# Autodesk Inventor assembly: Cover Optical Camera Only
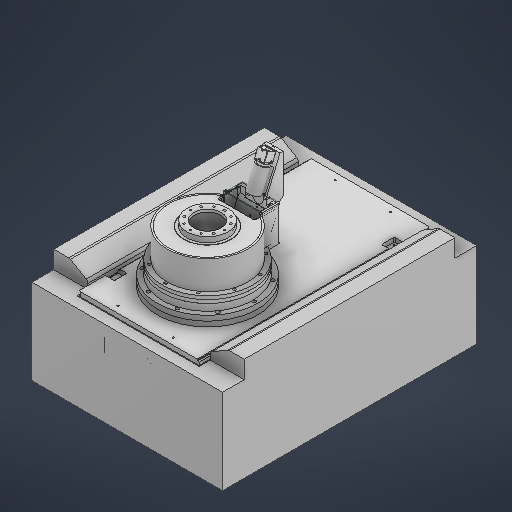
[picture p0: Inventor's stored thumbnail of the model, 512x512]
Saved by Autodesk Inventor 2025 (Build 290162000, 162)
## iProperties
Created: 2025-02-04
Part Number: Cover Optical Camera Only
Document SubType Name: Assembly
Designer: mayhe
Author: mayhe
## Documents named in this file (18)
- C:\Users\mayhe\OneDrive\Documents\GitHub\In-situ-monitoring-of-powder-bed-fusion-additive-manufacturing\system_development\Mithril\v0.2\Model\Cover Optical Camera Only.iam
- C:\Users\mayhe\OneDrive\Documents\GitHub\In-situ-monitoring-of-powder-bed-fusion-additive-manufacturing\system_development\Mithril\v0.2\Model\Cover (Optical Camera).ipt
- C:\Users\mayhe\OneDrive\Documents\GitHub\In-situ-monitoring-of-powder-bed-fusion-additive-manufacturing\system_development\Mithril\v0.2\Model\300mm Housing 1.ipt
- C:\Users\mayhe\OneDrive\Documents\GitHub\In-situ-monitoring-of-powder-bed-fusion-additive-manufacturing\system_development\Mithril\v0.2\Model\Cylinder Spacer Optical Camera.ipt
- C:\Users\mayhe\OneDrive\Documents\GitHub\In-situ-monitoring-of-powder-bed-fusion-additive-manufacturing\system_development\Mithril\v0.2\Model\Cylinder Segment\Cylinder Slidey Bit Housings\Cylinder Slidey Bit Housing Camera only v0.2.ipt
- C:\Users\mayhe\OneDrive\Documents\GitHub\In-situ-monitoring-of-powder-bed-fusion-additive-manufacturing\system_development\Mithril\v0.2\Model\300mm housing 2 Camera.ipt
- C:\Users\mayhe\OneDrive\Documents\GitHub\In-situ-monitoring-of-powder-bed-fusion-additive-manufacturing\system_development\Mithril\v0.2\Model\Cylinder Segment\Cylinder Segment Camera Only\C .Replace - Face.ipt
- C:\Users\mayhe\OneDrive\Documents\GitHub\In-situ-monitoring-of-powder-bed-fusion-additive-manufacturing\system_development\Mithril\v0.2\Model\Cylinder Segment\Cylinder Segment Camera Only.ipt
- C:\Users\mayhe\OneDrive\Documents\GitHub\In-situ-monitoring-of-powder-bed-fusion-additive-manufacturing\system_development\Mithril\v0.2\Model\Cylinder Segment\Cylinder Segment Camera Only\C .Replace - 10.ipt
- C:\Users\mayhe\OneDrive\Documents\GitHub\In-situ-monitoring-of-powder-bed-fusion-additive-manufacturing\system_development\Mithril\v0.2\Model\Cylinder Segment\Cylinder Segment  Camera only v0.2.ipt
- C:\Users\mayhe\OneDrive\Documents\GitHub\In-situ-monitoring-of-powder-bed-fusion-additive-manufacturing\system_development\Mithril\v0.2\Model\Cylinder Segment Holder.ipt
- C:\Users\mayhe\OneDrive\Documents\GitHub\In-situ-monitoring-of-powder-bed-fusion-additive-manufacturing\system_development\Mithril\v0.2\Model\Camera Bracket.ipt
- C:\Users\mayhe\OneDrive\Documents\GitHub\In-situ-monitoring-of-powder-bed-fusion-additive-manufacturing\system_development\Mithril\v0.2\Model\flircamera+lens.ipt
- C:\Users\mayhe\OneDrive\Documents\GitHub\In-situ-monitoring-of-powder-bed-fusion-additive-manufacturing\system_development\Mithril\v0.2\Model\Printer Body Camera Only.ipt
- C:\Users\mayhe\OneDrive\Documents\GitHub\In-situ-monitoring-of-powder-bed-fusion-additive-manufacturing\system_development\Mithril\v0.2\Model\substrate plate.ipt
- C:\Users\mayhe\OneDrive\Documents\GitHub\In-situ-monitoring-of-powder-bed-fusion-additive-manufacturing\system_development\Mithril\v0.2\Model\Welding Glass.ipt
- C:\Users\mayhe\OneDrive\Documents\GitHub\In-situ-monitoring-of-powder-bed-fusion-additive-manufacturing\system_development\Mithril\v0.2\Model\Cover^2.ipt
- C:\Users\mayhe\OneDrive\Documents\GitHub\In-situ-monitoring-of-powder-bed-fusion-additive-manufacturing\system_development\Mithril\v0.2\Model\cover^3.ipt
## Components (16 placed, 16 different names)
1. Cover (Optical Camera):1 — Rotational:5, Mate:5, Mate:6, Mate:7
2. 300mm Housing 1:1 — Rotational:5, Rotational:11
3. 300mm housing 2 Camera:2 — Rotational:11, Rotational:12
4. Cylinder Spacer Optical Camera:1 — Rotational:12, Rotational:13
5. Printer Body Camera Only:1 — Mate:5, Mate:6, Mate:7, Rotational:20
6. Cylinder Segment  Camera only v0.2:1 — Rotational:13, Rotational:14, Rotational:15, Rotational:17, Mate:10
7. Cylinder Slidey Bit Housing Camera only v0.2:1 — Rotational:14, Rotational:18, Flush:2, Mate:11
8. C .Replace - Face:1 — Rotational:16
9. C .Replace - 10:2 — Rotational:15, Rotational:16
10. Cylinder Segment Holder:1 — Rotational:17
11. Camera Bracket:1 — Rotational:18, Rotational:21, Mate:8, Mate:9, Flush:1
12. substrate plate:1 — Rotational:20
13. flircamera+lens:1 — Rotational:21
14. Welding Glass:1 — Mate:8, Mate:9, Flush:1
15. Cover^2:1 — Mate:10, Flush:2, Mate:11, Rotational:22
16. cover^3:1 — Rotational:22
## Relationships (21: RevoluteJoint 12, Mate 7, Flush 2)
- Rotational:5 [RevoluteJoint]: Cover (Optical Camera):1 ↔ 300mm Housing 1:1
- Rotational:11 [RevoluteJoint]: 300mm Housing 1:1 ↔ 300mm housing 2 Camera:2
- Rotational:12 [RevoluteJoint]: 300mm housing 2 Camera:2 ↔ Cylinder Spacer Optical Camera:1
- Mate:5: Cover (Optical Camera):1 ↔ Printer Body Camera Only:1
- Mate:6: Cover (Optical Camera):1 ↔ Printer Body Camera Only:1
- Mate:7: Cover (Optical Camera):1 ↔ Printer Body Camera Only:1
- Rotational:13 [RevoluteJoint]: Cylinder Spacer Optical Camera:1 ↔ Cylinder Segment  Camera only v0.2:1
- Rotational:14 [RevoluteJoint]: Cylinder Segment  Camera only v0.2:1 ↔ Cylinder Slidey Bit Housing Camera only v0.2:1
- Rotational:15 [RevoluteJoint]: Cylinder Segment  Camera only v0.2:1 ↔ C .Replace - 10:2
- Rotational:16 [RevoluteJoint]: C .Replace - Face:1 ↔ C .Replace - 10:2
- Rotational:17 [RevoluteJoint]: Cylinder Segment  Camera only v0.2:1 ↔ Cylinder Segment Holder:1
- Rotational:18 [RevoluteJoint]: Cylinder Slidey Bit Housing Camera only v0.2:1 ↔ Camera Bracket:1
- Rotational:20 [RevoluteJoint]: Printer Body Camera Only:1 ↔ substrate plate:1
- Rotational:21 [RevoluteJoint]: Camera Bracket:1 ↔ flircamera+lens:1
- Mate:8 (0.25 mm): Camera Bracket:1 ↔ Welding Glass:1
- Mate:9: Camera Bracket:1 ↔ Welding Glass:1
- Flush:1 (-30 mm): Camera Bracket:1 ↔ Welding Glass:1
- Mate:10: Cylinder Segment  Camera only v0.2:1 ↔ Cover^2:1
- Flush:2: Cylinder Slidey Bit Housing Camera only v0.2:1 ↔ Cover^2:1
- Mate:11 (2 mm): Cylinder Slidey Bit Housing Camera only v0.2:1 ↔ Cover^2:1
- Rotational:22 [RevoluteJoint]: Cover^2:1 ↔ cover^3:1
